# Autodesk Inventor assembly: gripper
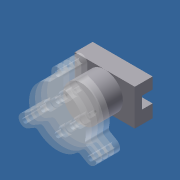
[picture p0: Inventor's stored thumbnail of the model, 180x180]
Saved by Autodesk Inventor 2012 (Build 160160000, 160)
## iProperties
Created: 2012-07-09
Part Number: gripper
Document SubType Name: Assembly
Designer: Ed
Author: Ed
## Documents named in this file (4)
- C:\Users\Ed\Documents\masters\Mechanical\Gripper\gripper.iam
- C:\Users\Ed\Documents\masters\Mechanical\Gripper\gripper.ipt
- C:\Users\Ed\Documents\masters\Mechanical\Gripper\acrylic gripper plate assy.iam
- C:\Users\Ed\Documents\masters\Mechanical\Gripper\IRB120 plate assy.iam
## Components (3 placed, 3 different names)
1. acrylic gripper plate assy:1 [sub-assembly] — Insert:1, Insert:2, Insert:3, Insert:4
2. gripper:1 — Insert:1, Insert:4
3. IRB120 plate assy:1 [sub-assembly] — Insert:2, Insert:3
## Relationships (4: Insert 4)
- Insert:1: acrylic gripper plate assy:1 ↔ gripper:1
- Insert:2: acrylic gripper plate assy:1 ↔ IRB120 plate assy:1
- Insert:3: acrylic gripper plate assy:1 ↔ IRB120 plate assy:1
- Insert:4: acrylic gripper plate assy:1 ↔ gripper:1
